# Autodesk Inventor assembly: whackAtDesignCam
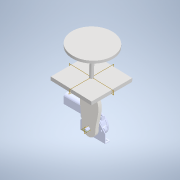
[picture p0: Inventor's stored thumbnail of the model, 180x180]
Saved by Autodesk Inventor 2020.2 (Build 242310000, 310)
## iProperties
Created: 2020-01-12
Part Number: whackAtDesignCam
Document SubType Name: Assembly
Designer: robst
Author: robst
## Documents named in this file (6)
- C:\git\CAD-Development\robSteele\2020BallTriggerMechanism\whackAtDesignCam.iam
- C:\git\CAD-Development\robSteele\2020BallTriggerMechanism\am-2235a Snow Blower Motor With Hex Shaft.iam
- C:\git\CAD-Development\robSteele\2020BallTriggerMechanism\Disc Cam3.ipt
- C:\git\CAD-Development\robSteele\2020BallTriggerMechanism\am-2373 Snow Blower Motor Mount.ipt
- C:\git\CAD-Development\robSteele\2020LongRobotBase\ballPlate.ipt
- C:\git\CAD-Development\robSteele\2020LongRobotBase\tableForBall.ipt
## Components (5 placed, 5 different names)
1. am-2235a Snow Blower Motor With Hex Shaft:1 [sub-assembly] — Insert:1, Insert:2, Flush:2, Flush:3, Mate:1, Mate:2
2. Disc Cam:1 — Flush:1, Mate:1, Mate:2
3. am-2373 Snow Blower Motor Mount:1 — Insert:1, Insert:2
4. ballPlate:1 — Insert:3
5. tableForBall:1 — Flush:1, Flush:2, Insert:3, Flush:3
## Relationships (8: Insert 3, Flush 3, Mate 2)
- Insert:1: am-2235a Snow Blower Motor With Hex Shaft:1 ↔ am-2373 Snow Blower Motor Mount:1
- Insert:2: am-2235a Snow Blower Motor With Hex Shaft:1 ↔ am-2373 Snow Blower Motor Mount:1
- Flush:1: Disc Cam:1 ↔ tableForBall:1
- Flush:2: am-2235a Snow Blower Motor With Hex Shaft:1 ↔ tableForBall:1
- Insert:3 (101.6 mm): ballPlate:1 ↔ tableForBall:1
- Flush:3 (-152.4 mm): am-2235a Snow Blower Motor With Hex Shaft:1 ↔ tableForBall:1
- Mate:1: am-2235a Snow Blower Motor With Hex Shaft:1 ↔ Disc Cam:1
- Mate:2: am-2235a Snow Blower Motor With Hex Shaft:1 ↔ Disc Cam:1
